# Autodesk Inventor assembly: powerTransferWithRoundbeltAndServo
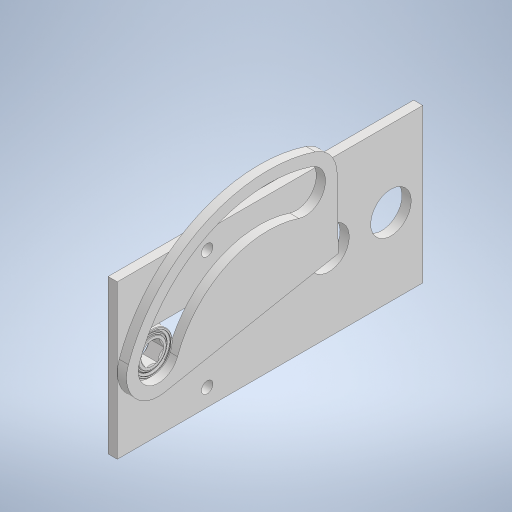
[picture p0: Inventor's stored thumbnail of the model, 512x512]
Saved by Autodesk Inventor 2023 (Build 270158000, 158)
## iProperties
Created: 2022-09-25
Part Number: powerTransferWithRoundbeltAndServo
Document SubType Name: Assembly
Designer: deli
Author: deli
## Documents named in this file (4)
- C:\Users\deli\OneDrive - Eastside Preparatory School\FTC\8103-power-play\CAD\powerTransferWithRoundbeltAndServo.iam
- C:\Users\deli\OneDrive - Eastside Preparatory School\FTC\8103-power-play\CAD\motorPlate.ipt
- C:\Users\deli\OneDrive - Eastside Preparatory School\FTC\8103-power-play\CAD\PulleyMover.ipt
- C:\Users\deli\OneDrive - Eastside Preparatory School\FTC\8103-power-play\CAD\FTC-parts\goBILDA\1611-0514-4008.ipt
## Components (3 placed, 3 different names)
1. motorPlate:1 — Mate:1, Mate:2, Mate:3, Mate:5
2. PulleyMover:1 — Mate:1, Mate:2, Mate:4
3. 1611-0514-4008:1 — Mate:3, Mate:4, Mate:5
## Relationships (5: Mate 5)
- Mate:1: motorPlate:1 ↔ PulleyMover:1
- Mate:2: motorPlate:1 ↔ PulleyMover:1
- Mate:3 (7 mm): motorPlate:1 ↔ 1611-0514-4008:1
- Mate:4 (40.3466 mm): PulleyMover:1 ↔ 1611-0514-4008:1
- Mate:5: motorPlate:1 ↔ 1611-0514-4008:1
